# Autodesk Inventor assembly: x ASY human dummy 01
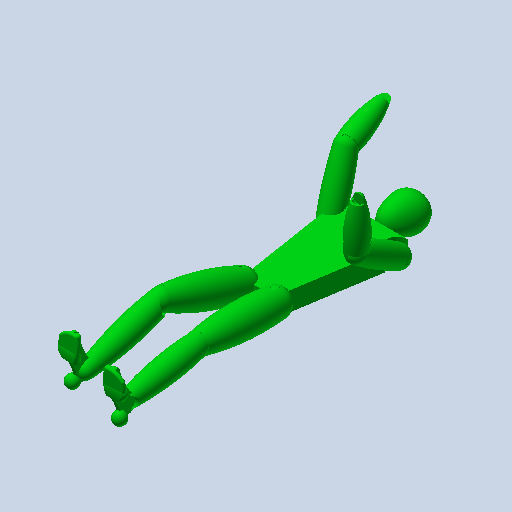
[picture p0: Inventor's stored thumbnail of the model, 512x512]
Saved by Autodesk Inventor 2024.2 (Build 282272000, 272)
## iProperties
Created: 2018-05-21
Part Number: x ASY human dummy 01
Material: Типовые
Document SubType Name: Assembly
Designer: admin
Stock Number: x ASY human dummy 01
Author: admin
Revision Number: 1
## Documents named in this file (12)
- C:\Users\admin\My Drive (bigstupidbeast@gmail.com)\Inventor\Nadyim\CAD\33 degree straight\dummi\human 01\x ASY human dummy 0.iam
- C:\Users\admin\My Drive (bigstupidbeast@gmail.com)\Inventor\Nadyim\CAD\33 degree straight\dummi\human 01\shoulder joint.ipt
- C:\Users\admin\My Drive (bigstupidbeast@gmail.com)\Inventor\Nadyim\CAD\33 degree straight\dummi\human 01\Shoulder parametric.ipt
- C:\Users\admin\My Drive (bigstupidbeast@gmail.com)\Inventor\Nadyim\CAD\33 degree straight\dummi\human 01\body parametric.ipt
- C:\Users\admin\My Drive (bigstupidbeast@gmail.com)\Inventor\Nadyim\CAD\33 degree straight\dummi\human 01\feet parametric.ipt
- C:\Users\admin\My Drive (bigstupidbeast@gmail.com)\Inventor\Nadyim\CAD\33 degree straight\dummi\human 01\Forearm.ipt
- C:\Users\admin\My Drive (bigstupidbeast@gmail.com)\Inventor\Nadyim\CAD\33 degree straight\dummi\human 01\Elbow.ipt
- C:\Users\admin\My Drive (bigstupidbeast@gmail.com)\Inventor\Nadyim\CAD\33 degree straight\dummi\human 01\Hip.ipt
- C:\Users\admin\My Drive (bigstupidbeast@gmail.com)\Inventor\Nadyim\CAD\33 degree straight\dummi\human 01\upper leg.ipt
- C:\Users\admin\My Drive (bigstupidbeast@gmail.com)\Inventor\Nadyim\CAD\33 degree straight\dummi\human 01\shank.ipt
- C:\Users\admin\My Drive (bigstupidbeast@gmail.com)\Inventor\Nadyim\CAD\33 degree straight\dummi\human 01\feet parametric_MIR.ipt
- C:\Users\admin\My Drive (bigstupidbeast@gmail.com)\Inventor\Nadyim\CAD\33 degree straight\dummi\human 01\Head.ipt
## Components (18 placed, 11 different names)
1. shoulder joint:1 — С поворотом:1, С поворотом:9
2. Shoulder parametric:1 — С поворотом:1, С поворотом:3
3. body parametric:1 — Заподлицо:2, С поворотом:9, Заподлицо:7, Заподлицо:8, С поворотом:10, С поворотом:14, С поворотом:15, Совмещение:1, Заподлицо:10
4. feet parametric:1 — С поворотом:20
5. Forearm:1 — С поворотом:2
6. Elbow:1 — С поворотом:2, С поворотом:3
7. Hip:1 — С поворотом:14, С поворотом:19
8. upper leg:1 — С поворотом:19, С поворотом:17
9. upper leg:2 — С поворотом:18, С поворотом:16
10. Hip:2 — С поворотом:15, С поворотом:18
11. shank:1 — С поворотом:16, С поворотом:20
12. shank:2 — С поворотом:17, С поворотом:21
13. shoulder joint:2 — С поворотом:10, С поворотом:11
14. Shoulder parametric:2 — С поворотом:11, С поворотом:13
15. Elbow:2 — С поворотом:12, С поворотом:13
16. Forearm:2 — С поворотом:12
17. feet parametric_MIR:1 — С поворотом:21
18. Head:1 — Заподлицо:9, Совмещение:1, Заподлицо:10
## Relationships (22: RevoluteJoint 16, Flush 5, Mate 1)
- С поворотом:1 [RevoluteJoint]: shoulder joint:1 ↔ Shoulder parametric:1
- Заподлицо:2 [Flush]: body parametric:1
- С поворотом:2 [RevoluteJoint]: Forearm:1 ↔ Elbow:1
- С поворотом:3 [RevoluteJoint]: Shoulder parametric:1 ↔ Elbow:1
- С поворотом:9 [RevoluteJoint]: shoulder joint:1 ↔ body parametric:1
- Заподлицо:7 [Flush]: body parametric:1
- Заподлицо:8 [Flush]: body parametric:1
- С поворотом:10 [RevoluteJoint]: body parametric:1 ↔ shoulder joint:2
- С поворотом:11 [RevoluteJoint]: shoulder joint:2 ↔ Shoulder parametric:2
- С поворотом:12 [RevoluteJoint]: Elbow:2 ↔ Forearm:2
- С поворотом:13 [RevoluteJoint]: Shoulder parametric:2 ↔ Elbow:2
- С поворотом:14 [RevoluteJoint]: body parametric:1 ↔ Hip:1
- С поворотом:15 [RevoluteJoint]: body parametric:1 ↔ Hip:2
- С поворотом:19 [RevoluteJoint]: Hip:1 ↔ upper leg:1
- С поворотом:18 [RevoluteJoint]: upper leg:2 ↔ Hip:2
- С поворотом:16 [RevoluteJoint]: upper leg:2 ↔ shank:1
- С поворотом:17 [RevoluteJoint]: upper leg:1 ↔ shank:2
- С поворотом:20 [RevoluteJoint]: feet parametric:1 ↔ shank:1
- С поворотом:21 [RevoluteJoint]: shank:2 ↔ feet parametric_MIR:1
- Заподлицо:9 [Flush]: Head:1
- Совмещение:1 [Mate] (100 mm): body parametric:1 ↔ Head:1
- Заподлицо:10 [Flush]: body parametric:1 ↔ Head:1
